# Autodesk Inventor assembly: button
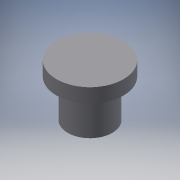
[picture p0: Inventor's stored thumbnail of the model, 180x180]
Saved by Autodesk Inventor 2016 SP2 (Build 200236200, 236)
## iProperties
Created: 2017-09-04
Part Number: button
Document SubType Name: Assembly
Designer: Kartikye
Author: Kartikye
## Documents named in this file (4)
- D:\Documents\cs294\keyboard\button.iam
- D:\Documents\cs294\keyboard\button_bottom.ipt
- D:\Documents\cs294\keyboard\button_part2.ipt
- D:\Documents\cs294\keyboard\button_part3.ipt
## Components (3 placed, 3 different names)
1. button_bottom:1 — Insert:2
2. button_part2:1 — Insert:1, Insert:2
3. button_part3:1 — Insert:1
## Relationships (2: Insert 2)
- Insert:1: button_part2:1 ↔ button_part3:1
- Insert:2: button_bottom:1 ↔ button_part2:1
